# Autodesk Inventor assembly: FullAssembly
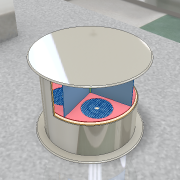
[picture p0: Inventor's stored thumbnail of the model, 180x180]
Saved by Autodesk Inventor 2018 (Build 220112000, 112)
## iProperties
Created: 2017-12-09
Part Number: FullAssembly
Document SubType Name: Assembly
Designer: Udara Wanasinghe
Author: Udara Wanasinghe
## Documents named in this file (3)
- D:\Documents\FIT\Hardware Project\Perfect\FullAssembly.iam
- D:\Documents\FIT\Hardware Project\Perfect\OuterCover.ipt
- D:\Documents\FIT\Hardware Project\Perfect\WaterproofCoverNRotatingPart.iam
## Components (2 placed, 2 different names)
1. OuterCover:1 — Insert:1, Flush:1
2. WaterproofCoverNRotatingPart:1 [sub-assembly] — Insert:1, Flush:1
## Relationships (2: Insert 1, Flush 1)
- Insert:1: OuterCover:1 ↔ WaterproofCoverNRotatingPart:1
- Flush:1: OuterCover:1 ↔ WaterproofCoverNRotatingPart:1
